# Autodesk Inventor assembly: Shock Cartridge
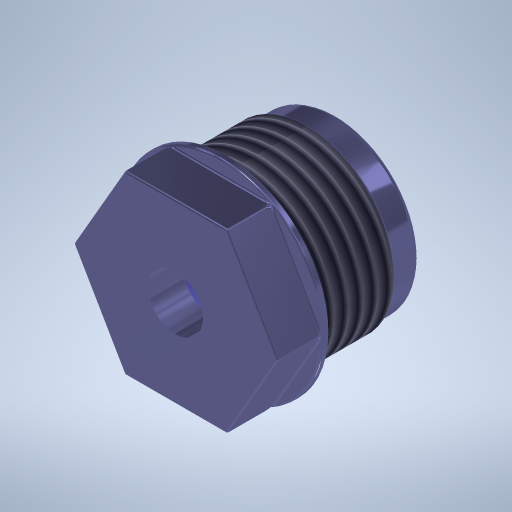
[picture p0: Inventor's stored thumbnail of the model, 512x512]
Saved by Autodesk Inventor 2023.1 (Build 271208000, 208)
## iProperties
Created: 2019-12-02
Part Number: Shock Cartridge
Document SubType Name: Assembly
Designer: Jopa
Author: Jopa
## Documents named in this file (5)
- C:\Users\Arzum Naz Doğaner\OneDrive\Masaüstü\HUDSON süspansiyon\Shock Cartridge.iam
- C:\Users\Arzum Naz Doğaner\OneDrive\Masaüstü\HUDSON süspansiyon\Shock Cartridge.ipt
- C:\Users\Arzum Naz Doğaner\OneDrive\Masaüstü\HUDSON süspansiyon\O-Ring.ipt
- C:\Users\Arzum Naz Doğaner\OneDrive\Masaüstü\HUDSON süspansiyon\Shock Cartridge Spacer.ipt
- C:\Users\Arzum Naz Doğaner\OneDrive\Masaüstü\HUDSON süspansiyon\Shock Cartridge Cover.ipt
## Components (5 placed, 4 different names)
1. Shock Cartridge:1 — Mate:1, Mate:2, Mate:3, Mate:4, Mate:5, Mate:6
2. O-Ring:1 — Mate:1, Mate:2, Flush:1
3. Shock Cartridge Spacer:1 — Mate:3, Flush:1, Flush:2
4. Shock Cartridge Cover:1 — Mate:5, Mate:6
5. O-Ring:2 — Mate:4, Flush:2
## Relationships (8: Mate 6, Flush 2)
- Mate:1: Shock Cartridge:1 ↔ O-Ring:1
- Mate:2: Shock Cartridge:1 ↔ O-Ring:1
- Mate:3: Shock Cartridge:1 ↔ Shock Cartridge Spacer:1
- Flush:1: O-Ring:1 ↔ Shock Cartridge Spacer:1
- Mate:4: Shock Cartridge:1 ↔ O-Ring:2
- Flush:2: Shock Cartridge Spacer:1 ↔ O-Ring:2
- Mate:5: Shock Cartridge:1 ↔ Shock Cartridge Cover:1
- Mate:6: Shock Cartridge:1 ↔ Shock Cartridge Cover:1
